# Autodesk Inventor assembly: test
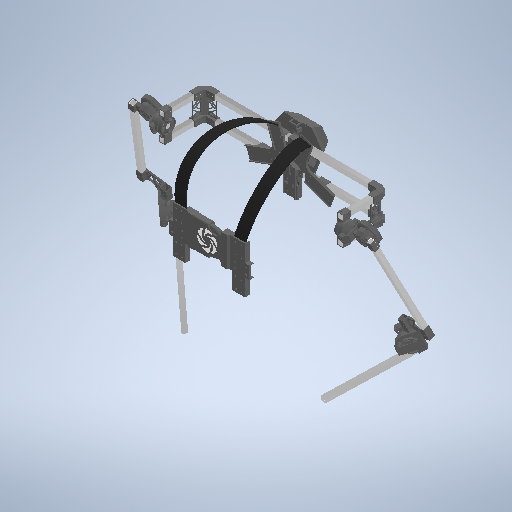
[picture p0: Inventor's stored thumbnail of the model, 512x512]
Saved by Autodesk Inventor 2026.1 (Build 301233020, 233B)
## iProperties
Created: 2026-02-01
Part Number: test
Document SubType Name: Assembly
Designer: hibik
Author: hibik
## Documents named in this file (26)
- C:\Users\hibik\Documents\Robomech\HR\controller\hard\body\Assy_body.iam
- C:\Users\hibik\Documents\Robomech\HR\controller\hard\body\body_size.ipt
- C:\Users\hibik\Documents\Robomech\HR\controller\hard\body\volume_upper.iam
- C:\Users\hibik\Documents\Robomech\HR\controller\hard\body\90_deg.ipt
- C:\Users\hibik\Documents\Robomech\HR\controller\hard\body\pipe_sholder_90deg2pitch.ipt
- C:\Users\hibik\Documents\Robomech\HR\controller\hard\body\volume_under.iam
- C:\Users\hibik\Documents\Robomech\HR\controller\hard\body\pipe_sholder_pitch245deg.ipt
- C:\Users\hibik\Documents\Robomech\HR\controller\hard\body\45_deg_right.ipt
- C:\Users\hibik\Documents\Robomech\HR\controller\hard\body\volume_case_under.ipt
- C:\Users\hibik\Documents\Robomech\HR\controller\hard\body\pipe_elbow2hand.ipt
- C:\Users\hibik\Documents\Robomech\HR\controller\hard\body\pipe_back.ipt
- C:\Users\hibik\Documents\Robomech\HR\controller\hard\body\volume_handle.ipt
- C:\Users\hibik\Documents\Robomech\HR\controller\hard\body\volume_connection.ipt
- C:\Users\hibik\Documents\Robomech\HR\controller\hard\body\pole_setter.ipt
- C:\Users\hibik\Documents\Robomech\HR\controller\hard\body\45_deg_left.ipt
- C:\Users\hibik\Documents\Robomech\HR\controller\hard\body\back_base.ipt
- C:\Users\hibik\Documents\Robomech\HR\controller\hard\body\back_base_MIR.ipt
- C:\Users\hibik\Documents\Robomech\HR\controller\hard\body\buckle_female.ipt
- C:\Users\hibik\Documents\Robomech\HR\controller\hard\body\buckle_male.ipt
- C:\Users\hibik\Documents\Robomech\HR\controller\hard\LOGO.ipt
- C:\Users\hibik\Documents\Robomech\HR\controller\hard\body\back_board_setter.ipt
- C:\Users\hibik\Documents\Robomech\HR\controller\hard\handle_right\battery_box.ipt
- C:\Users\hibik\Documents\Robomech\HR\controller\hard\body\board.ipt
- C:\Users\hibik\Documents\Robomech\HR\controller\hard\body\back_board_setter_cover.ipt
- C:\Users\hibik\Documents\Robomech\HR\controller\hard\body\back_battery_case.ipt
- C:\Users\hibik\Documents\Robomech\HR\controller\hard\body\belt.ipt
## Components (43 placed, 25 different names)
1. body_size:1
2. 90_deg:1 — 挿入:4, 挿入:5, 角度:3, 角度:4, 挿入:37, 角度:30
3. pipe_sholder_90deg2pitch:1 — 挿入:4, 角度:3, 挿入:11, 角度:9
4. pipe_sholder_90deg2pitch:2 — 挿入:5, 角度:4
5. volume_under:1 [sub-assembly] — 挿入:11, 角度:9, 挿入:64
6. pipe_sholder_pitch245deg:1 — 挿入:46, 角度:36, 挿入:60, 角度:48
7. 90_deg:2 — 挿入:36, 角度:29, 挿入:61, 角度:49
8. pipe_sholder_90deg2pitch:3
9. pipe_sholder_90deg2pitch:4
10. volume_under:4 [sub-assembly] — 挿入:38
11. pipe_sholder_pitch245deg:4 — 挿入:56, 角度:44, 挿入:62, 角度:50
12. 45_deg_right:1 — 挿入:27, 角度:22, 挿入:46, 角度:36
13. volume_case_under:1 — 挿入:27, 挿入:28, 角度:22
14. volume_upper:6 [sub-assembly] — 挿入:28, 挿入:30, 角度:24
15. pipe_elbow2hand:2 — 挿入:30, 角度:24
16. volume_case_under:2 — 挿入:63, 角度:51
17. volume_upper:7 [sub-assembly]
18. pipe_elbow2hand:3
19. pipe_back:1 — メイト:1, フラッシュ:1, メイト:2, 挿入:36, 角度:29, 挿入:37, 角度:30, 挿入:65, 角度:53, フラッシュ:5, メイト:4
20. volume_handle:1 — 挿入:38, 挿入:57, 角度:45
21. volume_handle:2 — 挿入:52, 角度:41, 挿入:64
22. volume_case_under:3 — 挿入:53, 挿入:54, 角度:52
23. volume_handle:3 — 挿入:54, 挿入:55, 角度:43
24. pole_setter:1 — 挿入:55, 角度:43, 挿入:56, 角度:44
25. volume_handle:4 — 挿入:50, 挿入:59, 角度:47
26. pole_setter:2 — 挿入:59, 角度:47, 挿入:60, 角度:48
27. volume_case_under:4 — 挿入:50, 挿入:58, 角度:46
28. volume_connection:3 — 挿入:52, 角度:41, 挿入:53, 角度:52
29. volume_connection:4 — 挿入:57, 角度:45, 挿入:58, 角度:46
30. pipe_back:2 — 挿入:61, 角度:49, 挿入:66, 角度:54, 角度:55
31. 45_deg_left:1 — 挿入:62, 角度:50, 挿入:63, 角度:51
32. back_base:1 — 挿入:65, 角度:53, メイト:10, メイト:13
33. back_base_MIR:1
34. buckle_female:1 — フラッシュ:2, フラッシュ:3, メイト:3, 対称度:1, フラッシュ:5, メイト:4, メイト:5, フラッシュ:7, メイト:11, メイト:12
35. buckle_male:1 — フラッシュ:2, フラッシュ:3, メイト:3, 対称度:1
36. LOGO:1 — フラッシュ:6, メイト:5, フラッシュ:7
37. back_board_setter:1 — 挿入:66, 角度:54, 挿入:67, フラッシュ:8, メイト:6, メイト:8, フラッシュ:11, メイト:9
38. battery_box:2 — 挿入:67, 角度:55
39. board:1
40. back_board_setter_cover:1 — フラッシュ:8, メイト:6, メイト:7, フラッシュ:9, フラッシュ:10
41. LOGO:2 — メイト:7, フラッシュ:9, フラッシュ:10
42. back_battery_case:1 — メイト:8, フラッシュ:11, メイト:9
43. belt:1 — メイト:10, メイト:11, メイト:12, メイト:13
## Relationships (83: Insert 32, Angle 26, Mate 13, Flush 11, Symmetry 1)
- 挿入:4 [Insert]: 90_deg:1 ↔ pipe_sholder_90deg2pitch:1
- 挿入:5 [Insert]: 90_deg:1 ↔ pipe_sholder_90deg2pitch:2
- 角度:3 [Angle] (0 deg): 90_deg:1 ↔ pipe_sholder_90deg2pitch:1
- 角度:4 [Angle] (0 deg): 90_deg:1 ↔ pipe_sholder_90deg2pitch:2
- 挿入:11 [Insert]: pipe_sholder_90deg2pitch:1 ↔ volume_under:1
- 角度:9 [Angle] (0 deg): pipe_sholder_90deg2pitch:1 ↔ volume_under:1
- [Insert]: 90_deg:2 ↔ pipe_sholder_90deg2pitch:3
- [Insert]: 90_deg:2 ↔ pipe_sholder_90deg2pitch:4
- [Angle] (0 deg): 90_deg:2 ↔ pipe_sholder_90deg2pitch:3
- [Angle] (0 deg): 90_deg:2 ↔ pipe_sholder_90deg2pitch:4
- [Insert]: pipe_sholder_90deg2pitch:3 ↔ volume_under:4
- [Angle] (0 deg): pipe_sholder_90deg2pitch:3 ↔ volume_under:4
- 挿入:27 [Insert]: 45_deg_right:1 ↔ volume_case_under:1
- 挿入:28 [Insert]: volume_case_under:1 ↔ volume_upper:6
- 挿入:30 [Insert]: volume_upper:6 ↔ pipe_elbow2hand:2
- 角度:22 [Angle] (0 deg): 45_deg_right:1 ↔ volume_case_under:1
- 角度:24 [Angle] (0 deg): volume_upper:6 ↔ pipe_elbow2hand:2
- [Insert]: volume_case_under:2 ↔ volume_upper:7
- [Insert]: volume_upper:7 ↔ pipe_elbow2hand:3
- [Angle] (0 deg): volume_upper:7 ↔ pipe_elbow2hand:3
- メイト:1 [Mate]: pipe_back:1
- フラッシュ:1 [Flush]: pipe_back:1
- メイト:2 [Mate]: pipe_back:1
- 挿入:36 [Insert]: 90_deg:2 ↔ pipe_back:1
- 角度:29 [Angle] (0 deg): 90_deg:2 ↔ pipe_back:1
- 挿入:37 [Insert]: 90_deg:1 ↔ pipe_back:1
- 角度:30 [Angle] (0 deg): 90_deg:1 ↔ pipe_back:1
- 挿入:38 [Insert]: volume_under:4 ↔ volume_handle:1
- 挿入:46 [Insert]: pipe_sholder_pitch245deg:1 ↔ 45_deg_right:1
- 角度:36 [Angle] (0 deg): pipe_sholder_pitch245deg:1 ↔ 45_deg_right:1
- 挿入:50 [Insert]: volume_handle:4 ↔ volume_case_under:4
- 挿入:52 [Insert]: volume_handle:2 ↔ volume_connection:3
- 角度:41 [Angle] (0 deg): volume_handle:2 ↔ volume_connection:3
- 挿入:53 [Insert]: volume_case_under:3 ↔ volume_connection:3
- 挿入:54 [Insert]: volume_case_under:3 ↔ volume_handle:3
- 挿入:55 [Insert]: volume_handle:3 ↔ pole_setter:1
- 角度:43 [Angle] (0 deg): volume_handle:3 ↔ pole_setter:1
- 挿入:56 [Insert]: pipe_sholder_pitch245deg:4 ↔ pole_setter:1
- 角度:44 [Angle] (0 deg): pipe_sholder_pitch245deg:4 ↔ pole_setter:1
- 挿入:57 [Insert]: volume_handle:1 ↔ volume_connection:4
- 角度:45 [Angle] (0 deg): volume_handle:1 ↔ volume_connection:4
- 挿入:58 [Insert]: volume_case_under:4 ↔ volume_connection:4
- 角度:46 [Angle] (0 deg): volume_case_under:4 ↔ volume_connection:4
- 挿入:59 [Insert]: volume_handle:4 ↔ pole_setter:2
- 角度:47 [Angle] (0 deg): volume_handle:4 ↔ pole_setter:2
- 挿入:60 [Insert]: pipe_sholder_pitch245deg:1 ↔ pole_setter:2
- 角度:48 [Angle] (0 deg): pipe_sholder_pitch245deg:1 ↔ pole_setter:2
- 挿入:61 [Insert]: 90_deg:2 ↔ pipe_back:2
- 角度:49 [Angle] (0 deg): 90_deg:2 ↔ pipe_back:2
- 挿入:62 [Insert]: pipe_sholder_pitch245deg:4 ↔ 45_deg_left:1
- 角度:50 [Angle] (0 deg): pipe_sholder_pitch245deg:4 ↔ 45_deg_left:1
- 挿入:63 [Insert]: volume_case_under:2 ↔ 45_deg_left:1
- 角度:51 [Angle] (0 deg): volume_case_under:2 ↔ 45_deg_left:1
- 挿入:64 [Insert]: volume_under:1 ↔ volume_handle:2
- 角度:52 [Angle] (0 deg): volume_case_under:3 ↔ volume_connection:3
- 挿入:65 [Insert]: pipe_back:1 ↔ back_base:1
- 角度:53 [Angle] (0 deg): pipe_back:1 ↔ back_base:1
- フラッシュ:2 [Flush]: buckle_female:1 ↔ buckle_male:1
- フラッシュ:3 [Flush]: buckle_female:1 ↔ buckle_male:1
- メイト:3 [Mate]: buckle_female:1 ↔ buckle_male:1
- 対称度:1 [Symmetry]: buckle_female:1 ↔ buckle_male:1
- フラッシュ:4 [Flush]
- フラッシュ:5 [Flush] (100 mm): pipe_back:1 ↔ buckle_female:1
- メイト:4 [Mate] (250 mm): pipe_back:1 ↔ buckle_female:1
- フラッシュ:6 [Flush]: LOGO:1
- メイト:5 [Mate]: buckle_female:1 ↔ LOGO:1
- フラッシュ:7 [Flush]: buckle_female:1 ↔ LOGO:1
- 挿入:66 [Insert]: pipe_back:2 ↔ back_board_setter:1
- 角度:54 [Angle] (180 deg): pipe_back:2 ↔ back_board_setter:1
- 挿入:67 [Insert]: back_board_setter:1 ↔ battery_box:2
- 角度:55 [Angle] (0 deg): pipe_back:2 ↔ battery_box:2
- フラッシュ:8 [Flush]: back_board_setter:1 ↔ back_board_setter_cover:1
- メイト:6 [Mate]: back_board_setter:1 ↔ back_board_setter_cover:1
- メイト:7 [Mate]: back_board_setter_cover:1 ↔ LOGO:2
- フラッシュ:9 [Flush]: back_board_setter_cover:1 ↔ LOGO:2
- フラッシュ:10 [Flush] (-57 mm): back_board_setter_cover:1 ↔ LOGO:2
- メイト:8 [Mate]: back_board_setter:1 ↔ back_battery_case:1
- フラッシュ:11 [Flush]: back_board_setter:1 ↔ back_battery_case:1
- メイト:9 [Mate]: back_board_setter:1 ↔ back_battery_case:1
- メイト:10 [Mate]: back_base:1 ↔ belt:1
- メイト:11 [Mate]: buckle_female:1 ↔ belt:1
- メイト:12 [Mate]: buckle_female:1 ↔ belt:1
- メイト:13 [Mate]: back_base:1 ↔ belt:1
## Named parameters: d78_d42 = 0 mm, d79_d43 = 0 mm, d80_d44 = 0 deg, d81_d45 = 0 deg, d89_d64 = 0 mm, d90_d65 = 0 deg, d106_d100 = 0 mm, d107_d101 = 0 mm, d109_d104 = 0 deg
